# Autodesk Inventor assembly: Suspension final
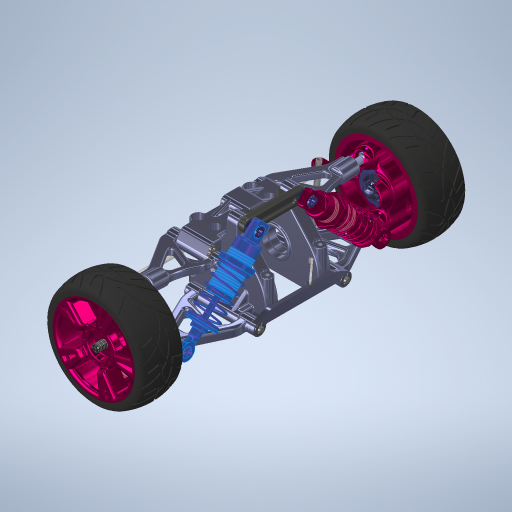
[picture p0: Inventor's stored thumbnail of the model, 512x512]
Saved by Autodesk Inventor 2023.1 (Build 271208000, 208)
## iProperties
Created: 2019-11-30
Part Number: Suspension final
Document SubType Name: Assembly
Designer: Jopa
Author: Jopa
## Documents named in this file (23)
- C:\Users\berke\Desktop\HUDSON-UKA\mechanics\Direksiyon Sistemi\Suspension + direksiyon final.iam
- C:\Users\berke\Desktop\HUDSON-UKA\mechanics\Direksiyon Sistemi\Front Side Plate R.ipt
- C:\Users\berke\Desktop\HUDSON-UKA\mechanics\Direksiyon Sistemi\Front Side Plate L.ipt
- C:\Users\berke\Desktop\HUDSON-UKA\mechanics\Direksiyon Sistemi\Front Upper Arm Mount.ipt
- C:\Users\berke\Desktop\HUDSON-UKA\mechanics\Direksiyon Sistemi\Front Shock Brace.ipt
- C:\Users\berke\Desktop\HUDSON-UKA\mechanics\Direksiyon Sistemi\Front Upper Arm.iam
- C:\Users\berke\Desktop\HUDSON-UKA\mechanics\Direksiyon Sistemi\Front Lower Arm.iam
- C:\Users\berke\Desktop\HUDSON-UKA\mechanics\Direksiyon Sistemi\Front Lower Arm Brace.ipt
- C:\Users\berke\Desktop\HUDSON-UKA\mechanics\Direksiyon Sistemi\Front Lower Hinge Pin.ipt
- C:\Users\berke\Desktop\HUDSON-UKA\mechanics\Direksiyon Sistemi\Front Upper Hinge Pin.ipt
- C:\Users\berke\Desktop\HUDSON-UKA\mechanics\Direksiyon Sistemi\E-Clip.ipt
- C:\Users\berke\Desktop\HUDSON-UKA\mechanics\Direksiyon Sistemi\Front Suspension Adjustment Clip.ipt
- C:\Users\berke\Desktop\HUDSON-UKA\mechanics\Direksiyon Sistemi\Shock Bushing.ipt
- C:\Users\berke\Desktop\HUDSON-UKA\mechanics\Direksiyon Sistemi\Shock Absorber.iam
- C:\Users\berke\Desktop\HUDSON-UKA\mechanics\Direksiyon Sistemi\Front Hub Carrier L.iam
- C:\Users\berke\Desktop\HUDSON-UKA\mechanics\Direksiyon Sistemi\Front Hub Carrier R.iam
- C:\Users\Arzum Naz Doğaner\OneDrive\Masaüstü\HUDSON süspansiyon\ISO 4762 - M3 x 20ISO.ipt
- C:\Users\Arzum Naz Doğaner\OneDrive\Masaüstü\HUDSON süspansiyon\ANSI B18.22.1 - No. 5 - narrow - Type B.ipt
- C:\Users\Arzum Naz Doğaner\OneDrive\Masaüstü\HUDSON süspansiyon\ISO 4035 - M3ISO.ipt
- C:\Users\Arzum Naz Doğaner\OneDrive\Masaüstü\HUDSON süspansiyon\ISO 4762 - M3 x 12ISO.ipt
- C:\Users\berke\Desktop\HUDSON-UKA\mechanics\Direksiyon Sistemi\alt şaft.ipt
- C:\Users\berke\Desktop\HUDSON-UKA\mechanics\Direksiyon Sistemi\üst şaft assembl.iam
- C:\Users\berke\Desktop\HUDSON-UKA\mechanics\Direksiyon Sistemi\servoya giden parca.ipt
## Components (46 placed, 22 different names)
1. Front Side Plate R:1 — Flush:1, Flush:2, Mate:1, Mate:2, Mate:4, Mate:6, Mate:7, Mate:12, Mate:13, Mate:14, Mate:59
2. Front Side Plate L:1 — Flush:1, Flush:2, Mate:1, Mate:3, Mate:5, Mate:8, Mate:9, Mate:17, Mate:18, Mate:58
3. Front Upper Arm Mount:1 — Mate:2, Mate:3, Mate:4, Mate:5, Mate:6, Mate:10, Mate:11, Mate:15, Mate:16, Mate:42, Mate:44, Insert:1, Insert:2, Insert:3, Insert:4
4. Front Shock Brace:1 — Mate:7, Mate:8, Mate:9, Mate:46, Mate:47, Mate:48, Mate:49
5. Front Upper Arm:1 [sub-assembly] — Mate:10, Mate:11, Mate:24, Flush:5, Mate:36, Mate:39, Mate:43, Mate:54
6. Front Lower Arm:1 [sub-assembly] — Mate:12, Mate:13, Mate:19, Mate:22, Mate:23, Mate:38, Mate:55, Mate:70
7. Front Upper Arm:2 [sub-assembly] — Mate:15, Mate:16, Mate:25, Flush:6, Mate:37, Mate:41, Mate:45, Mate:56
8. Front Lower Arm:2 [sub-assembly] — Mate:17, Mate:18, Mate:20, Mate:21, Mate:40, Mate:57, Mate:71
9. Front Lower Arm Brace:1 — Mate:19, Mate:20, Mate:23, Flush:3, Flush:4, Mate:34, Mate:35
10. Front Lower Hinge Pin:1 — Mate:21, Flush:4, Mate:26, Mate:31
11. Front Lower Hinge Pin:2 — Mate:22, Flush:3, Mate:27, Mate:32
12. Front Upper Hinge Pin:1 — Mate:24, Flush:5, Mate:28, Mate:33
13. Front Upper Hinge Pin:2 — Mate:25, Flush:6, Mate:29, Mate:30
14. E-Clip:1 — Mate:26, Mate:35
15. E-Clip:2 — Mate:27, Mate:34
16. E-Clip:3 — Mate:28, Mate:36
17. E-Clip:4 — Mate:29, Mate:37
18. E-Clip:5 — Mate:31, Mate:40
19. E-Clip:6 — Mate:33, Mate:39
20. E-Clip:7 — Mate:32, Mate:38
21. E-Clip:8 — Mate:30, Mate:41
22. Front Suspension Adjustment Clip:1 — Mate:42, Mate:43
23. Front Suspension Adjustment Clip:2 — Mate:44, Mate:45
24. Shock Bushing:1 — Mate:48, Mate:49, Mate:52, Mate:53, Mate:63
25. Shock Bushing:2 — Mate:46, Mate:47, Mate:50, Mate:51, Mate:62
26. Shock Absorber:1 [sub-assembly] — Mate:50, Mate:51, Mate:68, Mate:76
27. Shock Absorber:2 [sub-assembly] — Mate:52, Mate:53, Mate:69, Mate:77
28. Front Hub Carrier L:1 [sub-assembly] — Mate:54, Mate:55, Mate:79, Mate:81
29. Front Hub Carrier R:1 [sub-assembly] — Mate:56, Mate:57, Mate:78, Mate:80, Mate:82, Mate:83
30. ISO 4762 M3 x 20:1 — Mate:58, Mate:60, Mate:65
31. ISO 4762 M3 x 20:2 — Mate:59, Mate:61, Mate:64
32. Plain Washer (Inch) No. 5 - narrow - Type B:1 — Mate:60, Mate:63, Mate:67
33. Plain Washer (Inch) No. 5 - narrow - Type B:2 — Mate:61, Mate:62, Mate:66
34. ISO 4035 M3:1 — Mate:65, Mate:67
35. ISO 4035 M3:2 — Mate:64, Mate:66
36. ISO 4762 M3 x 12:1 — Mate:68, Mate:70, Mate:72, Mate:75
37. ISO 4762 M3 x 12:2 — Mate:69, Mate:71, Mate:73, Mate:74
38. Plain Washer (Inch) No. 5 - narrow - Type B:3 — Mate:72, Mate:75, Mate:76
39. Plain Washer (Inch) No. 5 - narrow - Type B:4 — Mate:73, Mate:74, Mate:77
40. ISO 4762 M3 x 12:3 — Insert:1
41. ISO 4762 M3 x 12:4 — Insert:2
42. ISO 4762 M3 x 12:5 — Insert:3
43. ISO 4762 M3 x 12:6 — Insert:4
44. alt şaft:1 — Mate:78, Mate:79, Mate:80, Mate:81
45. üst şaft assembl:1 [sub-assembly] — Mate:82, Mate:83, Mate:84, Mate:85
46. servoya giden parca:1 — Mate:84, Mate:85
## Relationships (95: Mate 85, Flush 6, Insert 4)
- Flush:1: Front Side Plate R:1 ↔ Front Side Plate L:1
- Flush:2: Front Side Plate R:1 ↔ Front Side Plate L:1
- Mate:1: Front Side Plate R:1 ↔ Front Side Plate L:1
- Mate:2: Front Side Plate R:1 ↔ Front Upper Arm Mount:1
- Mate:3: Front Side Plate L:1 ↔ Front Upper Arm Mount:1
- Mate:4: Front Side Plate R:1 ↔ Front Upper Arm Mount:1
- Mate:5: Front Side Plate L:1 ↔ Front Upper Arm Mount:1
- Mate:6 (2.3813 mm): Front Side Plate R:1 ↔ Front Upper Arm Mount:1
- Mate:7: Front Side Plate R:1 ↔ Front Shock Brace:1
- Mate:8: Front Side Plate L:1 ↔ Front Shock Brace:1
- Mate:9: Front Side Plate L:1 ↔ Front Shock Brace:1
- Mate:10: Front Upper Arm Mount:1 ↔ Front Upper Arm:1
- Mate:11: Front Upper Arm Mount:1 ↔ Front Upper Arm:1
- Mate:12: Front Side Plate R:1 ↔ Front Lower Arm:1
- Mate:13: Front Side Plate R:1 ↔ Front Lower Arm:1
- Mate:14: Front Side Plate R:1
- Mate:15: Front Upper Arm Mount:1 ↔ Front Upper Arm:2
- Mate:16: Front Upper Arm Mount:1 ↔ Front Upper Arm:2
- Mate:17: Front Side Plate L:1 ↔ Front Lower Arm:2
- Mate:18: Front Side Plate L:1 ↔ Front Lower Arm:2
- Mate:19: Front Lower Arm:1 ↔ Front Lower Arm Brace:1
- Mate:20: Front Lower Arm:2 ↔ Front Lower Arm Brace:1
- Mate:21: Front Lower Arm:2 ↔ Front Lower Hinge Pin:1
- Mate:22: Front Lower Arm:1 ↔ Front Lower Hinge Pin:2
- Mate:23: Front Lower Arm:1 ↔ Front Lower Arm Brace:1
- Flush:3: Front Lower Arm Brace:1 ↔ Front Lower Hinge Pin:2
- Flush:4: Front Lower Arm Brace:1 ↔ Front Lower Hinge Pin:1
- Mate:24: Front Upper Arm:1 ↔ Front Upper Hinge Pin:1
- Flush:5: Front Upper Arm:1 ↔ Front Upper Hinge Pin:1
- Mate:25: Front Upper Arm:2 ↔ Front Upper Hinge Pin:2
- Flush:6: Front Upper Arm:2 ↔ Front Upper Hinge Pin:2
- Mate:26: Front Lower Hinge Pin:1 ↔ E-Clip:1
- Mate:27: Front Lower Hinge Pin:2 ↔ E-Clip:2
- Mate:28: Front Upper Hinge Pin:1 ↔ E-Clip:3
- Mate:29: Front Upper Hinge Pin:2 ↔ E-Clip:4
- Mate:30: Front Upper Hinge Pin:2 ↔ E-Clip:8
- Mate:31: Front Lower Hinge Pin:1 ↔ E-Clip:5
- Mate:32: Front Lower Hinge Pin:2 ↔ E-Clip:7
- Mate:33: Front Upper Hinge Pin:1 ↔ E-Clip:6
- Mate:34: Front Lower Arm Brace:1 ↔ E-Clip:2
- Mate:35: Front Lower Arm Brace:1 ↔ E-Clip:1
- Mate:36: Front Upper Arm:1 ↔ E-Clip:3
- Mate:37: Front Upper Arm:2 ↔ E-Clip:4
- Mate:38: Front Lower Arm:1 ↔ E-Clip:7
- Mate:39: Front Upper Arm:1 ↔ E-Clip:6
- Mate:40: Front Lower Arm:2 ↔ E-Clip:5
- Mate:41: Front Upper Arm:2 ↔ E-Clip:8
- Mate:42: Front Upper Arm Mount:1 ↔ Front Suspension Adjustment Clip:1
- Mate:43: Front Upper Arm:1 ↔ Front Suspension Adjustment Clip:1
- Mate:44: Front Upper Arm Mount:1 ↔ Front Suspension Adjustment Clip:2
- Mate:45: Front Upper Arm:2 ↔ Front Suspension Adjustment Clip:2
- Mate:46: Front Shock Brace:1 ↔ Shock Bushing:2
- Mate:47: Front Shock Brace:1 ↔ Shock Bushing:2
- Mate:48: Front Shock Brace:1 ↔ Shock Bushing:1
- Mate:49: Front Shock Brace:1 ↔ Shock Bushing:1
- Mate:50: Shock Bushing:2 ↔ Shock Absorber:1
- Mate:51: Shock Bushing:2 ↔ Shock Absorber:1
- Mate:52: Shock Bushing:1 ↔ Shock Absorber:2
- Mate:53: Shock Bushing:1 ↔ Shock Absorber:2
- Mate:54: Front Upper Arm:1 ↔ Front Hub Carrier L:1
- Mate:55: Front Lower Arm:1 ↔ Front Hub Carrier L:1
- Mate:56: Front Upper Arm:2 ↔ Front Hub Carrier R:1
- Mate:57: Front Lower Arm:2 ↔ Front Hub Carrier R:1
- Mate:58: Front Side Plate L:1 ↔ ISO 4762 M3 x 20:1
- Mate:59: Front Side Plate R:1 ↔ ISO 4762 M3 x 20:2
- Mate:60: ISO 4762 M3 x 20:1 ↔ Plain Washer (Inch) No. 5 - narrow - Type B:1
- Mate:61: ISO 4762 M3 x 20:2 ↔ Plain Washer (Inch) No. 5 - narrow - Type B:2
- Mate:62: Shock Bushing:2 ↔ Plain Washer (Inch) No. 5 - narrow - Type B:2
- Mate:63: Shock Bushing:1 ↔ Plain Washer (Inch) No. 5 - narrow - Type B:1
- Mate:64: ISO 4762 M3 x 20:2 ↔ ISO 4035 M3:2
- Mate:65: ISO 4762 M3 x 20:1 ↔ ISO 4035 M3:1
- Mate:66: Plain Washer (Inch) No. 5 - narrow - Type B:2 ↔ ISO 4035 M3:2
- Mate:67: Plain Washer (Inch) No. 5 - narrow - Type B:1 ↔ ISO 4035 M3:1
- Mate:68: Shock Absorber:1 ↔ ISO 4762 M3 x 12:1
- Mate:69: Shock Absorber:2 ↔ ISO 4762 M3 x 12:2
- Mate:70: Front Lower Arm:1 ↔ ISO 4762 M3 x 12:1
- Mate:71: Front Lower Arm:2 ↔ ISO 4762 M3 x 12:2
- Mate:72: ISO 4762 M3 x 12:1 ↔ Plain Washer (Inch) No. 5 - narrow - Type B:3
- Mate:73: ISO 4762 M3 x 12:2 ↔ Plain Washer (Inch) No. 5 - narrow - Type B:4
- Mate:74: ISO 4762 M3 x 12:2 ↔ Plain Washer (Inch) No. 5 - narrow - Type B:4
- Mate:75: ISO 4762 M3 x 12:1 ↔ Plain Washer (Inch) No. 5 - narrow - Type B:3
- Mate:76: Shock Absorber:1 ↔ Plain Washer (Inch) No. 5 - narrow - Type B:3
- Mate:77: Shock Absorber:2 ↔ Plain Washer (Inch) No. 5 - narrow - Type B:4
- Insert:1: Front Upper Arm Mount:1 ↔ ISO 4762 M3 x 12:3
- Insert:2: Front Upper Arm Mount:1 ↔ ISO 4762 M3 x 12:4
- Insert:3: Front Upper Arm Mount:1 ↔ ISO 4762 M3 x 12:5
- Insert:4: Front Upper Arm Mount:1 ↔ ISO 4762 M3 x 12:6
- Mate:78: Front Hub Carrier R:1 ↔ alt şaft:1
- Mate:79: Front Hub Carrier L:1 ↔ alt şaft:1
- Mate:80: Front Hub Carrier R:1 ↔ alt şaft:1
- Mate:81: Front Hub Carrier L:1 ↔ alt şaft:1
- Mate:82: Front Hub Carrier R:1 ↔ üst şaft assembl:1
- Mate:83: Front Hub Carrier R:1 ↔ üst şaft assembl:1
- Mate:84: üst şaft assembl:1 ↔ servoya giden parca:1
- Mate:85: üst şaft assembl:1 ↔ servoya giden parca:1
